# Autodesk Inventor assembly: PCB Assembly
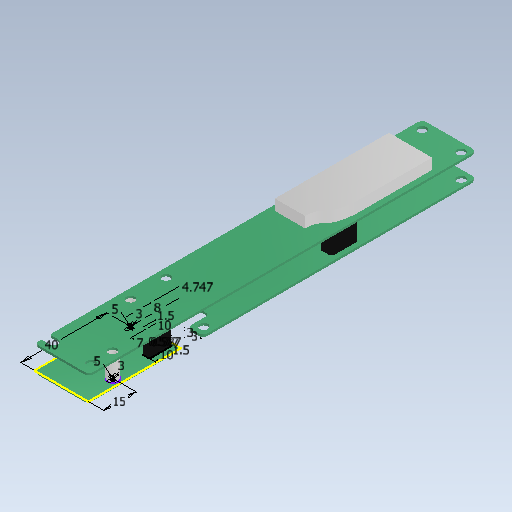
[picture p0: Inventor's stored thumbnail of the model, 512x512]
Saved by Autodesk Inventor 2021 (Build 250183000, 183)
## iProperties
Created: 2020-11-14
Part Number: PCB Assembly
Document SubType Name: Assembly
Designer: leoul
Author: leoul
## Documents named in this file (4)
- C:\Users\leoulgezu18\Desktop\Kinect 3D Modeling\Sub-assemblies\PCB Assembly.iam
- C:\Users\leoulgezu18\Desktop\Kinect 3D Modeling\Parts\PCB Large.ipt
- C:\Users\leoulgezu18\Desktop\Kinect 3D Modeling\Parts\PCB Medium.ipt
- C:\Users\leoulgezu18\Desktop\Kinect 3D Modeling\Parts\PCB Small.ipt
## Components (3 placed, 3 different names)
1. PCB Large:1 — Insert:1, Angle:1, Mate:1, Angle:2, Flush:1, Flush:2
2. PCB Medium:1 — Mate:1, Angle:2, Flush:1, Flush:2
3. PCB Small:1 — Insert:1, Angle:1
## Relationships (6: Angle 2, Flush 2, Insert 1, Mate 1)
- Insert:1: PCB Large:1 ↔ PCB Small:1
- Angle:1 (0 deg): PCB Large:1 ↔ PCB Small:1
- Mate:1: PCB Large:1 ↔ PCB Medium:1
- Angle:2 (0 deg): PCB Large:1 ↔ PCB Medium:1
- Flush:1: PCB Large:1 ↔ PCB Medium:1
- Flush:2: PCB Large:1 ↔ PCB Medium:1
